# Autodesk Inventor assembly: KOSZYK + ŁĄCZNIK
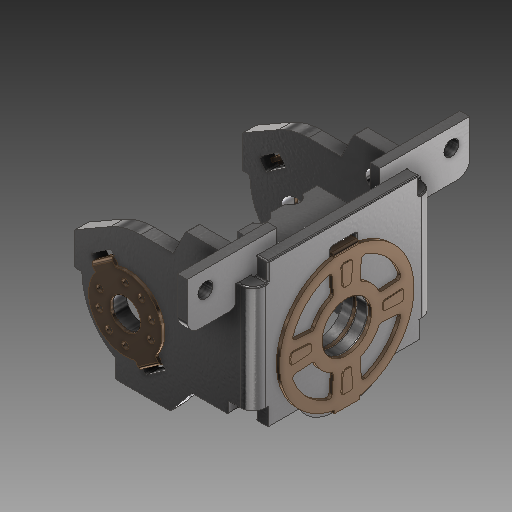
[picture p0: Inventor's stored thumbnail of the model, 512x512]
Saved by Autodesk Inventor 2017 SP1 (Build 210196100, 196)
## iProperties
Created: 2021-02-06
Part Number: KOSZYK + ŁĄCZNIK
Document SubType Name: Assembly
Designer: Napoleon
Author: Napoleon
## Documents named in this file (3)
- D:\PRYWATNE\PROJEKTY\POKÓJ\URZĄDZENIA PERYFERYJNE\DELL 1909Wf\KOSZYK + ŁĄCZNIK.iam
- D:\PRYWATNE\PROJEKTY\POKÓJ\URZĄDZENIA PERYFERYJNE\DELL 1909Wf\KOSZYK.iam
- D:\PRYWATNE\PROJEKTY\POKÓJ\URZĄDZENIA PERYFERYJNE\DELL 1909Wf\ŁĄCZNIK KOSZYKA.iam
## Components (2 placed, 2 different names)
1. KOSZYK:1 [sub-assembly] — Sztywne:1
2. ŁĄCZNIK KOSZYKA:1 [sub-assembly] — Sztywne:1
## Relationships (1: WeldJoint 1)
- Sztywne:1 [WeldJoint]: KOSZYK:1 ↔ ŁĄCZNIK KOSZYKA:1
